# Autodesk Inventor assembly: am-940a-6-HiGrip-
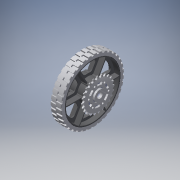
[picture p0: Inventor's stored thumbnail of the model, 180x180]
Saved by Autodesk Inventor 2016 (Build 200138000, 138)
## iProperties
Created: 2014-03-19
Part Number: am-940a-6-HiGrip-
Description: STEP AP214
Document SubType Name: Assembly
Designer: gus
Sending System: SolidWorks 2010
Preprocessor: SwSTEP 2.0
Title: 6-HiGrip-am-940aSTEP.STEP
Revision Number: ANY
## Documents named in this file (6)
- \\Mac\Home\Desktop\2016 robot cad\chassis\am-940a-6-HiGrip-.iam
- \\Mac\Home\Desktop\2016 robot cad\chassis\6 wheel Rev 4.ipt
- \\Mac\Home\Desktop\2016 robot cad\chassis\6 wheel tread II.ipt
- \\Mac\Home\Desktop\2016 robot cad\chassis\am-0077a-500 Key Hub r2.ipt
- \\Mac\Home\Desktop\2016 robot cad\chassis\24tsprocket.ipt
- \\Mac\Home\Desktop\2016 robot cad\chassis\shaftcollar.ipt
## Components (5 placed, 5 different names)
1. 6 wheel Rev 4_1 — Mate:1, Flush:1, Cylindrical:1, Mate:2
2. 6 wheel tread II_2 — Mate:1, Flush:1
3. am-0077a-500 Key Hub r2:1 — Cylindrical:1, Mate:2, Cylindrical:2, Mate:3, Mate:4, Rotational:1
4. 24tsprocket:1 — Cylindrical:2, Mate:3, Mate:4
5. shaftcollar:1 — Rotational:1
## Relationships (8: Mate 4, CylindricalJoint 2, Flush 1, RevoluteJoint 1)
- Mate:1: 6 wheel Rev 4_1 ↔ 6 wheel tread II_2
- Flush:1: 6 wheel Rev 4_1 ↔ 6 wheel tread II_2
- Cylindrical:1: 6 wheel Rev 4_1 ↔ am-0077a-500 Key Hub r2:1
- Mate:2: 6 wheel Rev 4_1 ↔ am-0077a-500 Key Hub r2:1
- Cylindrical:2: am-0077a-500 Key Hub r2:1 ↔ 24tsprocket:1
- Mate:3: am-0077a-500 Key Hub r2:1 ↔ 24tsprocket:1
- Mate:4: am-0077a-500 Key Hub r2:1 ↔ 24tsprocket:1
- Rotational:1 [RevoluteJoint]: am-0077a-500 Key Hub r2:1 ↔ shaftcollar:1
